# Autodesk Inventor assembly: Forearm
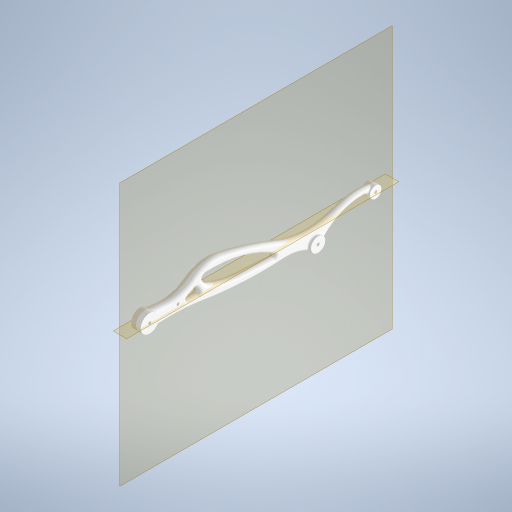
[picture p0: Inventor's stored thumbnail of the model, 512x512]
Saved by Autodesk Inventor 2023 (Build 270158000, 158)
## iProperties
Created: 2023-03-17
Part Number: Forearm
Document SubType Name: Assembly
Designer: valer
Author: valer
## Documents named in this file (2)
- C:\Users\LattePanda\Desktop\str1ker\description\models\src\Forearm.iam
- C:\Users\LattePanda\Desktop\str1ker\parts\Forearm.ipt
## Components (1 placed, 1 different names)
1. Forearm:1 — Mate:12, Mate:13, Mate:14
## Relationships (3: Mate 3)
- Mate:12: Forearm:1
- Mate:13: Forearm:1
- Mate:14: Forearm:1
